# Autodesk Inventor assembly: シールド先端
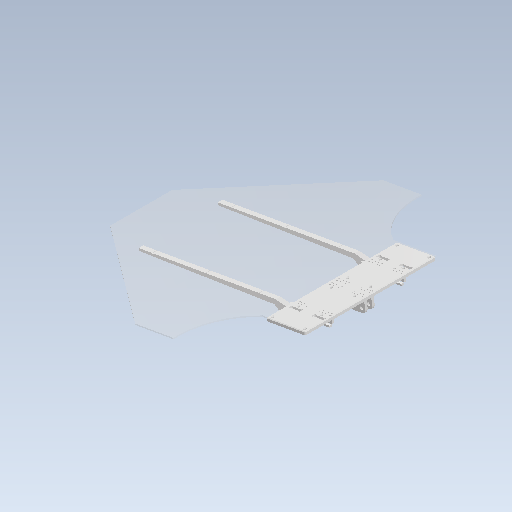
[picture p0: Inventor's stored thumbnail of the model, 512x512]
Saved by Autodesk Inventor 2020 (Build 240168000, 168)
## iProperties
Created: 2020-02-05
Part Number: シールド先端
Document SubType Name: Assembly
Designer: tanjihayato
Mass: 160.783 g
Surface Area: 1684.81 cm^2
Volume: 141.41 cm^3
Density: 1.137 g/cm^3
Author: tanjihayato
## Documents named in this file (7)
- \\Mac\Home\Documents\Inventor\2019お遊び機体\シールド先端.iam
- \\Mac\Home\Documents\Inventor\2019お遊び機体\シールド根本.ipt
- \\Mac\Home\Documents\Inventor\2019お遊び機体\シールド根本留め具.ipt
- \\Mac\Home\Documents\Inventor\2019お遊び機体\シールド板.ipt
- \\Mac\Home\Documents\Inventor\2019お遊び機体\シールド先端接続.ipt
- \\Mac\Home\Documents\Inventor\2019お遊び機体\シールド先端棒.ipt
- \\Mac\Home\Documents\Inventor\2019お遊び機体\シールド.ipt
## Components (9 placed, 6 different names)
1. シールド根本:1 — メイト:1, メイト:2, メイト:3, メイト:8, メイト:9
2. シールド根本留め具:1 — メイト:1, メイト:2, メイト:3, メイト:4, メイト:5, メイト:6, メイト:7
3. シールド根本:2 — メイト:4, メイト:5, メイト:6
4. シールド板:1 — メイト:7, メイト:8, メイト:9, フラッシュ:1, フラッシュ:2, メイト:10, メイト:11, メイト:12, メイト:13, 挿入:3, メイト:16
5. シールド先端接続:1 — フラッシュ:2, メイト:11, メイト:12, 挿入:2, メイト:14
6. シールド先端棒:1 — 挿入:2, メイト:14
7. シールド先端接続:2 — フラッシュ:1, メイト:10, メイト:13, 挿入:1, メイト:15
8. シールド先端棒:2 — 挿入:1, メイト:15
9. シールド:1 — 挿入:3, メイト:16
## Relationships (21: Mate 16, Insert 3, Flush 2)
- メイト:1 [Mate]: シールド根本:1 ↔ シールド根本留め具:1
- メイト:2 [Mate]: シールド根本:1 ↔ シールド根本留め具:1
- メイト:3 [Mate]: シールド根本:1 ↔ シールド根本留め具:1
- メイト:4 [Mate]: シールド根本留め具:1 ↔ シールド根本:2
- メイト:5 [Mate]: シールド根本留め具:1 ↔ シールド根本:2
- メイト:6 [Mate]: シールド根本留め具:1 ↔ シールド根本:2
- メイト:7 [Mate]: シールド根本留め具:1 ↔ シールド板:1
- メイト:8 [Mate]: シールド根本:1 ↔ シールド板:1
- メイト:9 [Mate]: シールド根本:1 ↔ シールド板:1
- フラッシュ:1 [Flush]: シールド板:1 ↔ シールド先端接続:2
- フラッシュ:2 [Flush]: シールド板:1 ↔ シールド先端接続:1
- メイト:10 [Mate]: シールド板:1 ↔ シールド先端接続:2
- メイト:11 [Mate]: シールド板:1 ↔ シールド先端接続:1
- メイト:12 [Mate]: シールド板:1 ↔ シールド先端接続:1
- メイト:13 [Mate]: シールド板:1 ↔ シールド先端接続:2
- 挿入:1 [Insert]: シールド先端接続:2 ↔ シールド先端棒:2
- 挿入:2 [Insert]: シールド先端接続:1 ↔ シールド先端棒:1
- メイト:14 [Mate]: シールド先端接続:1 ↔ シールド先端棒:1
- メイト:15 [Mate]: シールド先端接続:2 ↔ シールド先端棒:2
- 挿入:3 [Insert]: シールド板:1 ↔ シールド:1
- メイト:16 [Mate]: シールド板:1 ↔ シールド:1
